# Autodesk Inventor assembly: Drive Train Assembly
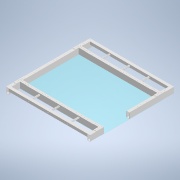
[picture p0: Inventor's stored thumbnail of the model, 180x180]
Saved by Autodesk Inventor 2020 (Build 240168000, 168)
## iProperties
Created: 2020-01-14
Part Number: Drive Train Assembly
Document SubType Name: Assembly
Designer: aidan
Author: aidan
## Documents named in this file (10)
- C:\Users\aidan\Desktop\T3 Robotics\Drive Train Assembly.iam
- C:\Users\aidan\Desktop\T3 Robotics\VerseFrame 28in.ipt
- C:\Users\aidan\Desktop\T3 Robotics\VerseFrame 30in.ipt
- C:\Users\aidan\Desktop\T3 Robotics\1x1 28in WChurro Holes.ipt
- C:\Users\aidan\Desktop\T3 Robotics\Churro 4in.ipt
- C:\Users\aidan\Desktop\T3 Robotics\Cut Lexan DriveTrain.ipt
- C:\Users\aidan\Desktop\T3 Robotics\TGusset Versa.ipt
- C:\Users\aidan\Desktop\T3 Robotics\VerseFrame 5in STOCK.ipt
- C:\Users\aidan\Desktop\T3 Robotics\VerseFrame 16in.ipt
- C:\Users\aidan\Desktop\T3 Robotics\VersaGusset 90o.ipt
## Components (18 placed, 9 different names)
1. VerseFrame 28in:1 — Mate:1, Flush:1, Flush:3, Flush:5, Mate:26, Mate:27, Flush:17, Flush:24, Mate:30, Flush:27, Flush:28, Flush:34
2. VerseFrame 28in:2 — Flush:2, Mate:2, Flush:3, Mate:25, Flush:25, Mate:31, Flush:29, Flush:30, Flush:31, Mate:33
3. VerseFrame 30in:1 — Mate:1, Flush:1, Flush:2, Mate:2, Flush:5, Flush:8, Flush:11, Flush:12, Mate:5, Mate:28, Mate:29, Flush:23, Flush:26
4. 1x1 28in WChurro Holes:2 — Flush:8, Mate:13, Mate:14, Mate:15
5. 1x1 28in WChurro Holes:3 — Flush:11, Flush:12, Mate:5, Mate:16, Mate:17, Mate:18, Mate:33
6. Churro 4in:1 — Flush:13, Flush:14, Mate:9, Mate:26
7. Churro 4in:2 — Flush:13, Mate:6
8. Churro 4in:3 — Flush:14, Mate:8
9. Churro 4in:4 — Mate:10, Flush:15
10. Churro 4in:5 — Mate:11, Flush:15, Flush:16
11. Churro 4in:6 — Mate:12, Flush:16, Mate:25
12. Cut Lexan DriveTrain:1 — Mate:27, Flush:17
13. TGusset Versa:1 — Mate:28, Flush:23, Flush:24
14. TGusset Versa:2 — Mate:29, Flush:25, Flush:26
15. TGusset Versa:4 — Flush:30, Flush:31, Flush:32, Mate:34
16. VerseFrame 5in STOCK:1 — Mate:30, Flush:27, Flush:28, Mate:32, Mate:35, Flush:33
17. VerseFrame 16in:1 — Mate:31, Mate:32, Flush:29, Flush:32, Mate:34
18. VersaGusset 90o:1 — Mate:35, Flush:33, Flush:34
## Relationships (56: Mate 32, Flush 24)
- Mate:1: VerseFrame 28in:1 ↔ VerseFrame 30in:1
- Flush:1: VerseFrame 28in:1 ↔ VerseFrame 30in:1
- Flush:2: VerseFrame 28in:2 ↔ VerseFrame 30in:1
- Mate:2: VerseFrame 28in:2 ↔ VerseFrame 30in:1
- Flush:3: VerseFrame 28in:1 ↔ VerseFrame 28in:2
- Flush:5 (-101.6 mm): VerseFrame 28in:1 ↔ VerseFrame 30in:1
- Flush:8: VerseFrame 30in:1 ↔ 1x1 28in WChurro Holes:2
- Flush:11: VerseFrame 30in:1 ↔ 1x1 28in WChurro Holes:3
- Flush:12: VerseFrame 30in:1 ↔ 1x1 28in WChurro Holes:3
- Mate:5: VerseFrame 30in:1 ↔ 1x1 28in WChurro Holes:3
- Flush:13: Churro 4in:1 ↔ Churro 4in:2
- Flush:14: Churro 4in:1 ↔ Churro 4in:3
- Mate:6: Churro 4in:2
- Mate:8: Churro 4in:3
- Mate:9: Churro 4in:1
- Mate:10: Churro 4in:4
- Mate:11: Churro 4in:5
- Mate:12: Churro 4in:6
- Flush:15: Churro 4in:4 ↔ Churro 4in:5
- Flush:16: Churro 4in:5 ↔ Churro 4in:6
- Mate:13: 1x1 28in WChurro Holes:2
- Mate:14: 1x1 28in WChurro Holes:2
- Mate:15: 1x1 28in WChurro Holes:2
- Mate:16: 1x1 28in WChurro Holes:3
- Mate:17: 1x1 28in WChurro Holes:3
- Mate:18: 1x1 28in WChurro Holes:3
- Mate:19
- Mate:20
- Mate:21
- Mate:22
- Mate:23
- Mate:24
- Mate:25: VerseFrame 28in:2 ↔ Churro 4in:6
- Mate:26: VerseFrame 28in:1 ↔ Churro 4in:1
- Mate:27: VerseFrame 28in:1 ↔ Cut Lexan DriveTrain:1
- Flush:17: VerseFrame 28in:1 ↔ Cut Lexan DriveTrain:1
- Mate:28: VerseFrame 30in:1 ↔ TGusset Versa:1
- Mate:29: VerseFrame 30in:1 ↔ TGusset Versa:2
- Flush:23: VerseFrame 30in:1 ↔ TGusset Versa:1
- Flush:24: VerseFrame 28in:1 ↔ TGusset Versa:1
- Flush:25: VerseFrame 28in:2 ↔ TGusset Versa:2
- Flush:26: VerseFrame 30in:1 ↔ TGusset Versa:2
- Mate:30: VerseFrame 28in:1 ↔ VerseFrame 5in STOCK:1
- Flush:27: VerseFrame 28in:1 ↔ VerseFrame 5in STOCK:1
- Flush:28: VerseFrame 28in:1 ↔ VerseFrame 5in STOCK:1
- Mate:31: VerseFrame 28in:2 ↔ VerseFrame 16in:1
- Mate:32 (228.6 mm): VerseFrame 5in STOCK:1 ↔ VerseFrame 16in:1
- Flush:29: VerseFrame 28in:2 ↔ VerseFrame 16in:1
- Flush:30: VerseFrame 28in:2 ↔ TGusset Versa:4
- Flush:31: VerseFrame 28in:2 ↔ TGusset Versa:4
- Flush:32: TGusset Versa:4 ↔ VerseFrame 16in:1
- Mate:33 (76.2 mm): VerseFrame 28in:2 ↔ 1x1 28in WChurro Holes:3
- Mate:34: TGusset Versa:4 ↔ VerseFrame 16in:1
- Mate:35: VerseFrame 5in STOCK:1 ↔ VersaGusset 90o:1
- Flush:33: VerseFrame 5in STOCK:1 ↔ VersaGusset 90o:1
- Flush:34: VerseFrame 28in:1 ↔ VersaGusset 90o:1
